# Autodesk Inventor assembly: Camera_Newcap_Holder_45Deg_5mm Assembly
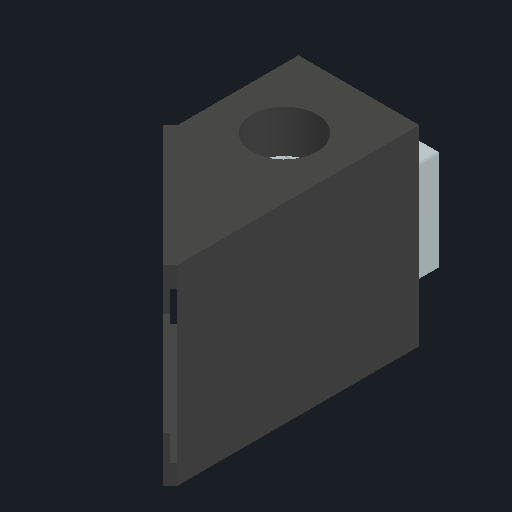
[picture p0: Inventor's stored thumbnail of the model, 512x512]
Saved by Autodesk Inventor 2026 (Build 300175000, 175)
## iProperties
Created: 2026-03-19
Part Number: Camera_Newcap_Holder_45Deg_5mm Assembly
Document SubType Name: Assembly
Designer: FiolkaLab
Author: FiolkaLab
## Documents named in this file (3)
- E:\Muaaz\Baseplate\Detection\Camera_Newcap_Holder_45Deg_5mm Assembly.iam
- E:\Muaaz\Baseplate\Detection\Camera\Camera Assembly with new Cap.iam
- E:\Muaaz\Baseplate\Detection\Camera Holder V2 BP Height and 45 Deg.ipt
## Components (2 placed, 2 different names)
1. Camera Assembly with new Cap:1 [sub-assembly] — Mate:1, Mate:2, Angle:1
2. Camera Holder V2 BP Height and 45 Deg:1 — Mate:1, Mate:2, Angle:1
## Relationships (3: Mate 2, Angle 1)
- Mate:1: Camera Assembly with new Cap:1 ↔ Camera Holder V2 BP Height and 45 Deg:1
- Mate:2: Camera Assembly with new Cap:1 ↔ Camera Holder V2 BP Height and 45 Deg:1
- Angle:1 (0 deg): Camera Assembly with new Cap:1 ↔ Camera Holder V2 BP Height and 45 Deg:1
